# Autodesk Inventor assembly: 276-1810-LARGE
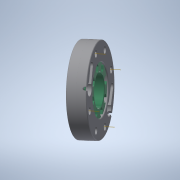
[picture p0: Inventor's stored thumbnail of the model, 180x180]
Saved by Autodesk Inventor 2020 (Build 240168000, 168)
## iProperties
Created: 2011-04-18
Part Number: 276-1810-LARGE
Material: 常规
Description: STEP AP203
Document SubType Name: Assembly
Designer: aresp
Sending System: SolidWorks 2010
Preprocessor: SwSTEP 2.0
Title: 276-1810-LARGE.STEP
Revision Number: ANY
## Documents named in this file (6)
- D:\vault\ncrCadLib\高级力学套件\276-1810-LARGE.iam
- D:\vault\ncrCadLib\高级力学套件\Reference Parts\276-1810-002.ipt
- D:\vault\ncrCadLib\高级力学套件\Reference Parts\276-1810-004.ipt
- D:\vault\ncrCadLib\高级力学套件\Reference Parts\276-1810-003.ipt
- C:\Users\aresp\Documents\Inventor\Content Center Files\R2020\zh-CN\防滑螺帽\防滑落幕.ipt
- C:\Users\aresp\Documents\Inventor\Content Center Files\R2020\zh-CN\Screw 8-32 x 0.750'' 五号\275-1006-001.ipt
## Components (11 placed, 5 different names)
1. 276-1810-002_3 — 配合:3, 配合:4
2. 276-1810-004_6 — 配合:1, 配合:2, 配合:5, 配合:10, 配合:11
3. 276-1810-003_10 — 配合:1, 配合:2, 配合:3, 配合:4, 配合:5, 配合:9
4. Screw 8-32 x 0.750'' 五号 275-1006-001:1 — 配合:10, 配合:11, 配合:8
5. 防滑螺帽 防滑落幕:1 — 配合:8, 配合:9
6. Screw 8-32 x 0.750'' 五号 275-1006-001:2
7. 防滑螺帽 防滑落幕:2
8. Screw 8-32 x 0.750'' 五号 275-1006-001:3
9. 防滑螺帽 防滑落幕:3
10. Screw 8-32 x 0.750'' 五号 275-1006-001:4
11. 防滑螺帽 防滑落幕:4
## Component patterns: (4 elements, first: Screw 8-32 x 0.750'' 五号 275-1006-001:1 + 防滑螺帽 防滑落幕:1)
## Relationships (9: Mate 9)
- 配合:1 [Mate]: 276-1810-004_6 ↔ 276-1810-003_10
- 配合:2 [Mate]: 276-1810-004_6 ↔ 276-1810-003_10
- 配合:3 [Mate]: 276-1810-002_3 ↔ 276-1810-003_10
- 配合:4 [Mate]: 276-1810-002_3 ↔ 276-1810-003_10
- 配合:5 [Mate]: 276-1810-004_6 ↔ 276-1810-003_10
- 配合:8 [Mate]: Screw 8-32 x 0.750'' 五号 275-1006-001:1 ↔ 防滑螺帽 防滑落幕:1
- 配合:9 [Mate]: 276-1810-003_10 ↔ 防滑螺帽 防滑落幕:1
- 配合:10 [Mate]: 276-1810-004_6 ↔ Screw 8-32 x 0.750'' 五号 275-1006-001:1
- 配合:11 [Mate]: 276-1810-004_6 ↔ Screw 8-32 x 0.750'' 五号 275-1006-001:1
